# Autodesk Inventor assembly: MechSwitch_Assembly
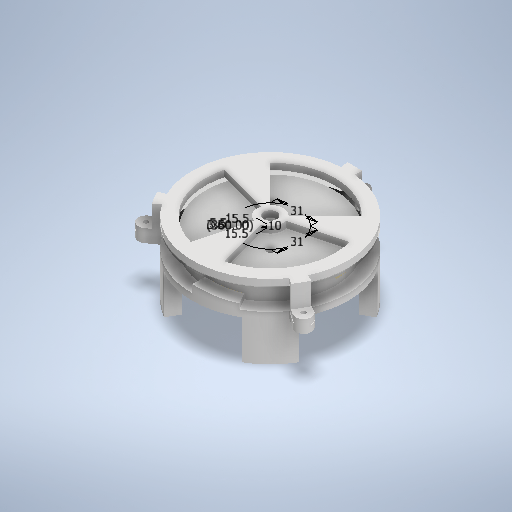
[picture p0: Inventor's stored thumbnail of the model, 512x512]
Saved by Autodesk Inventor 2025.1 (Build 291241000, 241)
## iProperties
Created: 2026-02-23
Part Number: MechSwitch_Assembly
Document SubType Name: Assembly
Designer: ryand
Author: ryand
## Documents named in this file (4)
- C:\Users\ryand\OneDrive\Documents\Inventor\TNG\Rotational_TENG\MechSwitch\MechSwitch_Assembly.iam
- C:\Users\ryand\OneDrive\Documents\Inventor\TNG\Rotational_TENG\MechSwitch\MechSwitch_DielecTop.ipt
- C:\Users\ryand\OneDrive\Documents\Inventor\TNG\Rotational_TENG\MechSwitch\MechSwitch_MotorBaseipt.ipt
- C:\Users\ryand\OneDrive\Documents\Grad Research\Rot_TENG_PCB\ResearchFocusSchematic\ResearchFocusSchem\ResearchFocusSchem\ResearchFocusSchem.ipt
## Components (3 placed, 3 different names)
1. MechSwitch_DielecTop:1 — Mate:1
2. MechSwitch_MotorBaseipt:1 — Mate:1, Rigid:1
3. ResearchFocusSchem:1 — Rigid:1
## Relationships (2: Mate 1, WeldJoint 1)
- Mate:1: MechSwitch_DielecTop:1 ↔ MechSwitch_MotorBaseipt:1
- Rigid:1 [WeldJoint]: MechSwitch_MotorBaseipt:1 ↔ ResearchFocusSchem:1
